# Autodesk Inventor assembly: TubeLensWAdapter
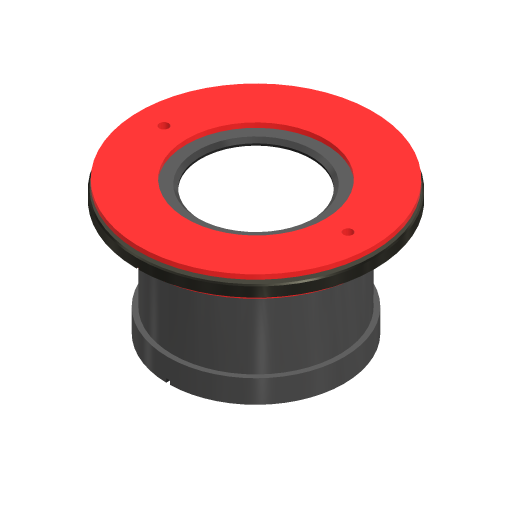
[picture p0: Inventor's stored thumbnail of the model, 512x512]
Saved by Autodesk Inventor 2023 (Build 270158000, 158)
## iProperties
Created: 2023-06-23
Part Number: TubeLensWAdapter
Document SubType Name: Assembly
Designer: nvladi
Author: nvladi
## Documents named in this file (4)
- C:\Users\Public\GitHub-public\benchtop-hardware\Benchtop\CAD-model-Inventor\mesoSPIM\detection_path\Mitutoyo\TubeLensWAdapter.iam
- C:\Users\Public\GitHub-public\benchtop-hardware\Benchtop\CAD-model-Inventor\library\Thorlabs\optics\ITL200.ipt
- C:\Users\Public\GitHub-public\benchtop-hardware\Benchtop\custom-parts\detection-accessories\Mitutoyo-MT1(tube-lens)-SM2-adapter\Adapter-MitutoyoMT1-SM2.ipt
- C:\Users\Public\GitHub-public\benchtop-hardware\Benchtop\CAD-model-Inventor\library\Thorlabs\accessoires\SM2RR.ipt
## Components (3 placed, 3 different names)
1. ITL200:1 — Insert:1
2. Adapter-MitutoyoMT1-SM2:1 — Insert:1, Insert:2
3. SM2RR:1 — Insert:2
## Relationships (2: Insert 2)
- Insert:1 (1 mm): ITL200:1 ↔ Adapter-MitutoyoMT1-SM2:1
- Insert:2 (3 mm): Adapter-MitutoyoMT1-SM2:1 ↔ SM2RR:1
